# Autodesk Inventor assembly: Assembly1
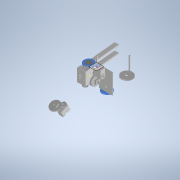
[picture p0: Inventor's stored thumbnail of the model, 180x180]
Saved by Autodesk Inventor 2020.2 (Build 242310000, 310)
## iProperties
Created: 2022-10-31
Part Number: Assembly1
Document SubType Name: Assembly
Designer: Administrator
Author: Administrator
## Documents named in this file (15)
- C:\Users\Administrator\Documents\kamuy2\Assembly1.iam
- C:\Users\Administrator\Documents\kamuy2\Parts\Part1.ipt
- C:\Users\Administrator\Documents\kamuy2\Parts\x-540_idle.ipt
- C:\Users\Administrator\Documents\kamuy2\Parts\XW540.N105.I101.ipt
- C:\Users\Administrator\Documents\kamuy2\Parts\GEABP1.0-80-10-A-20-KFC30-K3_Autodesk_Inventor_2020_20221101\AIS2020\GEABP1_0-80-10-A-20-KFC30-K3.iam
- C:\Users\Administrator\Documents\kamuy2\Parts\GEABP1.0-32-10-A-12-KFC22-K3_Autodesk_Inventor_2020_20221101\AIS2020\GEABP1_0-32-10-A-12-KFC22-K3.iam
- C:\Users\Administrator\Documents\kamuy2\Parts\Part2.ipt
- C:\Users\Administrator\Documents\kamuy2\Parts\BGHK6800VV-20_Autodesk_Inventor_2020_20221102\AIS2020\BGHK6800VV-20.iam
- C:\Users\Administrator\Documents\kamuy2\Parts\GEABP1.0-70-10-B-10-KFC30-K3_Autodesk_Inventor_2020_20221102\AIS2020\GEABP1_0-70-10-B-10-KFC30-K3.iam
- C:\Users\Administrator\Documents\kamuy2\Parts\Part7.ipt
- C:\Users\Administrator\Documents\kamuy2\Parts\HTPA23S3M060-A-P10_Autodesk_Inventor_2020_20221104\AIS2020\HTPA23S3M060-A-P10.iam
- C:\Users\Administrator\Documents\kamuy2\Parts\BGHK6800VV-30_Autodesk_Inventor_2020_20221102\AIS2020\BGHK6800VV-30.iam
- C:\Users\Administrator\Documents\kamuy2\Part9.ipt
- C:\Users\Administrator\Documents\kamuy2\Parts\GEYK1.0-70-10-B-10K_Autodesk_Inventor_2020_20221114\AIS2020\GEYK1_0-70-10-B-10K.iam
- C:\Users\Administrator\Documents\kamuy2\Part2.ipt
## Components (28 placed, 13 different names)
1. Part1:1 — フラッシュ:1, メイト:1, フラッシュ:14, メイト:13, フラッシュ:15
2. x-540_idle:1 — メイト:4, メイト:5, フラッシュ:36, メイト:65, フラッシュ:45, メイト:71, メイト:72, フラッシュ:47
3. XW540.N105.I101:1 — フラッシュ:1, メイト:1, メイト:2, メイト:3, フラッシュ:14, メイト:70
4. GEABP1_0-32-10-A-12-KFC22-K3:1 [sub-assembly] — メイト:2, メイト:3, フラッシュ:22
5. GEABP1_0-32-10-A-12-KFC22-K3:2 [sub-assembly] — メイト:4, メイト:5, フラッシュ:50
6. Part2:1
7. x-540_idle:2
8. GEABP1_0-32-10-A-12-KFC22-K3:3 [sub-assembly] — フラッシュ:24
9. GEABP1_0-80-10-A-20-KFC30-K3:4 [sub-assembly]
10. BGHK6800VV-20:1 [sub-assembly] — メイト:13, フラッシュ:15, メイト:24, メイト:67, メイト:70
11. GEABP1_0-70-10-B-10-KFC30-K3:1 [sub-assembly] — フラッシュ:22, メイト:24
12. GEABP1_0-70-10-B-10-KFC30-K3:3 [sub-assembly] — フラッシュ:24
13. Part7:1
14. x-540_idle:3 — フラッシュ:36, フラッシュ:45, メイト:71, フラッシュ:48
15. GEABP1_0-32-10-A-12-KFC22-K3:4 [sub-assembly] — フラッシュ:46
16. Part7:2 — フラッシュ:40
17. Part7:3 — メイト:56, メイト:60, メイト:69
18. HTPA23S3M060-A-P10:1 [sub-assembly] — メイト:56, メイト:68
19. BGHK6800VV-30:1 [sub-assembly] — メイト:60, フラッシュ:42, フラッシュ:43, フラッシュ:44, メイト:73
20. Part9:1 — フラッシュ:39, フラッシュ:41, メイト:62
21. Part9:2 — フラッシュ:39, フラッシュ:40, フラッシュ:41
22. Part7:4 — メイト:67
23. BGHK6800VV-30:2 [sub-assembly] — フラッシュ:42, メイト:62, メイト:65, フラッシュ:49, メイト:74
24. BGHK6800VV-30:3 [sub-assembly] — フラッシュ:43, フラッシュ:44, メイト:68, フラッシュ:49
25. GEYK1_0-70-10-B-10K:1 [sub-assembly] — メイト:69, フラッシュ:46
26. Part2:2 — メイト:72, フラッシュ:47, メイト:73, フラッシュ:48
27. GEYK1_0-70-10-B-10K:2 [sub-assembly] — フラッシュ:50, メイト:74
28. GEYK1_0-70-10-B-10K:3 [sub-assembly]
## Relationships (41: Mate 23, Flush 18)
- フラッシュ:1 [Flush]: Part1:1 ↔ XW540.N105.I101:1
- メイト:1 [Mate]: Part1:1 ↔ XW540.N105.I101:1
- メイト:2 [Mate]: XW540.N105.I101:1 ↔ GEABP1_0-32-10-A-12-KFC22-K3:1
- メイト:3 [Mate]: XW540.N105.I101:1 ↔ GEABP1_0-32-10-A-12-KFC22-K3:1
- メイト:4 [Mate]: x-540_idle:1 ↔ GEABP1_0-32-10-A-12-KFC22-K3:2
- メイト:5 [Mate]: x-540_idle:1 ↔ GEABP1_0-32-10-A-12-KFC22-K3:2
- [Mate]: x-540_idle:2 ↔ GEABP1_0-32-10-A-12-KFC22-K3:3
- [Mate]: x-540_idle:2 ↔ GEABP1_0-32-10-A-12-KFC22-K3:3
- フラッシュ:14 [Flush]: Part1:1 ↔ XW540.N105.I101:1
- メイト:13 [Mate]: Part1:1 ↔ BGHK6800VV-20:1
- フラッシュ:15 [Flush]: Part1:1 ↔ BGHK6800VV-20:1
- フラッシュ:22 [Flush]: GEABP1_0-32-10-A-12-KFC22-K3:1 ↔ GEABP1_0-70-10-B-10-KFC30-K3:1
- メイト:24 [Mate]: BGHK6800VV-20:1 ↔ GEABP1_0-70-10-B-10-KFC30-K3:1
- フラッシュ:24 [Flush]: GEABP1_0-32-10-A-12-KFC22-K3:3 ↔ GEABP1_0-70-10-B-10-KFC30-K3:3
- [Mate]: x-540_idle:3 ↔ GEABP1_0-32-10-A-12-KFC22-K3:4
- [Mate]: x-540_idle:3 ↔ GEABP1_0-32-10-A-12-KFC22-K3:4
- フラッシュ:36 [Flush]: x-540_idle:1 ↔ x-540_idle:3
- メイト:56 [Mate]: Part7:3 ↔ HTPA23S3M060-A-P10:1
- フラッシュ:39 [Flush]: Part9:1 ↔ Part9:2
- フラッシュ:40 [Flush] (-10 mm): Part7:2 ↔ Part9:2
- フラッシュ:41 [Flush]: Part9:1 ↔ Part9:2
- メイト:60 [Mate]: Part7:3 ↔ BGHK6800VV-30:1
- フラッシュ:42 [Flush]: BGHK6800VV-30:1 ↔ BGHK6800VV-30:2
- メイト:62 [Mate] (1 mm): Part9:1 ↔ BGHK6800VV-30:2
- メイト:65 [Mate] (6.591 mm): x-540_idle:1 ↔ BGHK6800VV-30:2
- フラッシュ:43 [Flush]: BGHK6800VV-30:1 ↔ BGHK6800VV-30:3
- フラッシュ:44 [Flush]: BGHK6800VV-30:1 ↔ BGHK6800VV-30:3
- メイト:67 [Mate]: BGHK6800VV-20:1 ↔ Part7:4
- メイト:68 [Mate] (2 mm): HTPA23S3M060-A-P10:1 ↔ BGHK6800VV-30:3
- メイト:69 [Mate]: Part7:3 ↔ GEYK1_0-70-10-B-10K:1
- メイト:70 [Mate] (12.15 mm): XW540.N105.I101:1 ↔ BGHK6800VV-20:1
- フラッシュ:45 [Flush]: x-540_idle:1 ↔ x-540_idle:3
- メイト:71 [Mate]: x-540_idle:1 ↔ x-540_idle:3
- フラッシュ:46 [Flush]: GEABP1_0-32-10-A-12-KFC22-K3:4 ↔ GEYK1_0-70-10-B-10K:1
- メイト:72 [Mate]: x-540_idle:1 ↔ Part2:2
- フラッシュ:47 [Flush]: x-540_idle:1 ↔ Part2:2
- メイト:73 [Mate]: BGHK6800VV-30:1 ↔ Part2:2
- フラッシュ:48 [Flush]: x-540_idle:3 ↔ Part2:2
- フラッシュ:49 [Flush]: BGHK6800VV-30:2 ↔ BGHK6800VV-30:3
- フラッシュ:50 [Flush]: GEABP1_0-32-10-A-12-KFC22-K3:2 ↔ GEYK1_0-70-10-B-10K:2
- メイト:74 [Mate]: BGHK6800VV-30:2 ↔ GEYK1_0-70-10-B-10K:2
## Named parameters: d10_d5 = 0 mm, d11_d6 = 0 mm, d99_d5 = 0 mm, d100_d6 = 0 mm
